# Autodesk Inventor assembly: Waffling60-MX
(part 2 of 2)
56. Open CASCADE STEP translator 7.5 468
57. Open CASCADE STEP translator 7.5 469
58. Open CASCADE STEP translator 7.5 470
59. Open CASCADE STEP translator 7.5 471
60. Open CASCADE STEP translator 7.5 472
61. Open CASCADE STEP translator 7.5 473
62. Open CASCADE STEP translator 7.5 474
63. Open CASCADE STEP translator 7.5 475
64. Open CASCADE STEP translator 7.5 476
65. Open CASCADE STEP translator 7.5 477
66. Open CASCADE STEP translator 7.5 478
67. Open CASCADE STEP translator 7.5 479
68. Open CASCADE STEP translator 7.5 480
69. Open CASCADE STEP translator 7.5 481
70. Open CASCADE STEP translator 7.5 482
71. Open CASCADE STEP translator 7.5 483
72. Open CASCADE STEP translator 7.5 484
73. Open CASCADE STEP translator 7.5 485
74. Open CASCADE STEP translator 7.5 486
75. Open CASCADE STEP translator 7.5 487
76. Open CASCADE STEP translator 7.5 488
77. Open CASCADE STEP translator 7.5 489
78. Open CASCADE STEP translator 7.5 490
79. Open CASCADE STEP translator 7.5 491
80. Open CASCADE STEP translator 7.5 492
81. Open CASCADE STEP translator 7.5 493
82. Open CASCADE STEP translator 7.5 494
83. Open CASCADE STEP translator 7.5 495
84. Open CASCADE STEP translator 7.5 496
85. Open CASCADE STEP translator 7.5 497
86. Open CASCADE STEP translator 7.5 498
87. Open CASCADE STEP translator 7.5 499
88. Open CASCADE STEP translator 7.5 500
89. Open CASCADE STEP translator 7.5 501
90. Open CASCADE STEP translator 7.5 502
91. Open CASCADE STEP translator 7.5 503
92. Open CASCADE STEP translator 7.5 504
93. Open CASCADE STEP translator 7.5 505
94. Open CASCADE STEP translator 7.5 506
95. Open CASCADE STEP translator 7.5 507
96. Open CASCADE STEP translator 7.5 508
97. Open CASCADE STEP translator 7.5 509
98. Open CASCADE STEP translator 7.5 510
99. Open CASCADE STEP translator 7.5 511
100. Open CASCADE STEP translator 7.5 512
101. Open CASCADE STEP translator 7.5 513
102. Open CASCADE STEP translator 7.5 514
103. Open CASCADE STEP translator 7.5 515
104. Open CASCADE STEP translator 7.5 516
105. Open CASCADE STEP translator 7.5 517
106. Open CASCADE STEP translator 7.5 518
107. Open CASCADE STEP translator 7.5 519
108. Open CASCADE STEP translator 7.5 520
109. Open CASCADE STEP translator 7.5 521
110. Open CASCADE STEP translator 7.5 522
111. Open CASCADE STEP translator 7.5 523
112. Open CASCADE STEP translator 7.5 524
113. Open CASCADE STEP translator 7.5 525
114. Open CASCADE STEP translator 7.5 526
115. Open CASCADE STEP translator 7.5 527
116. Open CASCADE STEP translator 7.5 528
117. Open CASCADE STEP translator 7.5 529
118. Open CASCADE STEP translator 7.5 530
119. Open CASCADE STEP translator 7.5 531
120. Open CASCADE STEP translator 7.5 532
121. Open CASCADE STEP translator 7.5 533
122. Open CASCADE STEP translator 7.5 534
123. Open CASCADE STEP translator 7.5 535
124. Open CASCADE STEP translator 7.5 536
125. Open CASCADE STEP translator 7.5 537
126. Open CASCADE STEP translator 7.5 538
127. Open CASCADE STEP translator 7.5 539
128. Open CASCADE STEP translator 7.5 540
129. Open CASCADE STEP translator 7.5 541
130. Open CASCADE STEP translator 7.5 542
131. Open CASCADE STEP translator 7.5 543
132. Open CASCADE STEP translator 7.5 544
133. Open CASCADE STEP translator 7.5 545
134. Open CASCADE STEP translator 7.5 546
135. Open CASCADE STEP translator 7.5 547
136. Open CASCADE STEP translator 7.5 548
137. Open CASCADE STEP translator 7.5 549
138. Open CASCADE STEP translator 7.5 550
139. Open CASCADE STEP translator 7.5 551
140. Open CASCADE STEP translator 7.5 552
141. Open CASCADE STEP translator 7.5 553
142. Open CASCADE STEP translator 7.5 554
143. Open CASCADE STEP translator 7.5 555
144. Open CASCADE STEP translator 7.5 556
145. Open CASCADE STEP translator 7.5 557
146. Open CASCADE STEP translator 7.5 558
147. Open CASCADE STEP translator 7.5 559
148. Open CASCADE STEP translator 7.5 560
149. Open CASCADE STEP translator 7.5 561
150. Open CASCADE STEP translator 7.5 562
151. Open CASCADE STEP translator 7.5 563
152. Open CASCADE STEP translator 7.5 564
153. Open CASCADE STEP translator 7.5 565
154. Open CASCADE STEP translator 7.5 566
155. Open CASCADE STEP translator 7.5 567
156. Open CASCADE STEP translator 7.5 568
157. Open CASCADE STEP translator 7.5 569
158. Open CASCADE STEP translator 7.5 570
159. Open CASCADE STEP translator 7.5 571
160. Open CASCADE STEP translator 7.5 572
161. Open CASCADE STEP translator 7.5 573
162. Open CASCADE STEP translator 7.5 574
163. Open CASCADE STEP translator 7.5 575
164. Open CASCADE STEP translator 7.5 576
165. Open CASCADE STEP translator 7.5 577
166. Open CASCADE STEP translator 7.5 578
167. Open CASCADE STEP translator 7.5 579
168. Open CASCADE STEP translator 7.5 580
169. Open CASCADE STEP translator 7.5 581
170. Open CASCADE STEP translator 7.5 582
171. Open CASCADE STEP translator 7.5 583
172. Open CASCADE STEP translator 7.5 584
173. Open CASCADE STEP translator 7.5 585
174. Open CASCADE STEP translator 7.5 586
175. Open CASCADE STEP translator 7.5 587
176. Open CASCADE STEP translator 7.5 588
177. Open CASCADE STEP translator 7.5 589
178. Open CASCADE STEP translator 7.5 590
179. Open CASCADE STEP translator 7.5 591
180. Open CASCADE STEP translator 7.5 592
181. Open CASCADE STEP translator 7.5 593
182. Open CASCADE STEP translator 7.5 594
183. Open CASCADE STEP translator 7.5 595
184. Open CASCADE STEP translator 7.5 596
185. Open CASCADE STEP translator 7.5 597
186. Open CASCADE STEP translator 7.5 598
187. Open CASCADE STEP translator 7.5 599
188. Open CASCADE STEP translator 7.5 600
189. Open CASCADE STEP translator 7.5 601
190. Open CASCADE STEP translator 7.5 602
191. Open CASCADE STEP translator 7.5 603
192. Open CASCADE STEP translator 7.5 604
193. Open CASCADE STEP translator 7.5 605
194. Open CASCADE STEP translator 7.5 606
195. Open CASCADE STEP translator 7.5 607
196. Open CASCADE STEP translator 7.5 608
197. Open CASCADE STEP translator 7.5 609
198. Open CASCADE STEP translator 7.5 610
199. Open CASCADE STEP translator 7.5 611
200. Open CASCADE STEP translator 7.5 612
201. Open CASCADE STEP translator 7.5 613
202. Open CASCADE STEP translator 7.5 614
203. Open CASCADE STEP translator 7.5 615
204. Open CASCADE STEP translator 7.5 616
205. Open CASCADE STEP translator 7.5 617
206. Open CASCADE STEP translator 7.5 618
207. Open CASCADE STEP translator 7.5 619
208. Open CASCADE STEP translator 7.5 620
209. Open CASCADE STEP translator 7.5 621
210. Open CASCADE STEP translator 7.5 622
211. Open CASCADE STEP translator 7.5 623
212. Open CASCADE STEP translator 7.5 624
213. Open CASCADE STEP translator 7.5 625
214. Open CASCADE STEP translator 7.5 626
215. Open CASCADE STEP translator 7.5 627
216. Open CASCADE STEP translator 7.5 628
217. Open CASCADE STEP translator 7.5 629
218. Open CASCADE STEP translator 7.5 630
219. Open CASCADE STEP translator 7.5 631
220. Open CASCADE STEP translator 7.5 632
221. Open CASCADE STEP translator 7.5 633
222. Open CASCADE STEP translator 7.5 634
223. Open CASCADE STEP translator 7.5 635
224. Open CASCADE STEP translator 7.5 636
225. Open CASCADE STEP translator 7.5 637
226. Open CASCADE STEP translator 7.5 638
227. Open CASCADE STEP translator 7.5 639
228. Open CASCADE STEP translator 7.5 640
229. Open CASCADE STEP translator 7.5 641
230. Open CASCADE STEP translator 7.5 642
231. Open CASCADE STEP translator 7.5 643
232. Open CASCADE STEP translator 7.5 644
233. Open CASCADE STEP translator 7.5 645
234. Open CASCADE STEP translator 7.5 646
235. Open CASCADE STEP translator 7.5 647
236. Open CASCADE STEP translator 7.5 648
237. Open CASCADE STEP translator 7.5 649
238. Open CASCADE STEP translator 7.5 650
239. Open CASCADE STEP translator 7.5 651
240. Open CASCADE STEP translator 7.5 652
241. Open CASCADE STEP translator 7.5 653
242. Open CASCADE STEP translator 7.5 654
243. Open CASCADE STEP translator 7.5 655
244. Open CASCADE STEP translator 7.5 656
245. Open CASCADE STEP translator 7.5 657
246. Open CASCADE STEP translator 7.5 658
247. Open CASCADE STEP translator 7.5 659
248. Open CASCADE STEP translator 7.5 660
249. Open CASCADE STEP translator 7.5 661
250. Open CASCADE STEP translator 7.5 662
251. Open CASCADE STEP translator 7.5 663
252. Open CASCADE STEP translator 7.5 664
253. Open CASCADE STEP translator 7.5 665
254. Open CASCADE STEP translator 7.5 666
255. Open CASCADE STEP translator 7.5 667
256. Open CASCADE STEP translator 7.5 668
257. Open CASCADE STEP translator 7.5 669
258. Open CASCADE STEP translator 7.5 670
259. Open CASCADE STEP translator 7.5 671
260. Open CASCADE STEP translator 7.5 672
261. Open CASCADE STEP translator 7.5 673
262. Open CASCADE STEP translator 7.5 674
263. Open CASCADE STEP translator 7.5 675
264. Open CASCADE STEP translator 7.5 676
265. Open CASCADE STEP translator 7.5 677
266. Open CASCADE STEP translator 7.5 678
267. Open CASCADE STEP translator 7.5 679
268. Open CASCADE STEP translator 7.5 680
269. Open CASCADE STEP translator 7.5 681
270. Open CASCADE STEP translator 7.5 682
271. Open CASCADE STEP translator 7.5 683
272. Open CASCADE STEP translator 7.5 684
273. Open CASCADE STEP translator 7.5 685
274. Open CASCADE STEP translator 7.5 686
275. Open CASCADE STEP translator 7.5 687
276. Open CASCADE STEP translator 7.5 688
277. Open CASCADE STEP translator 7.5 689
278. Open CASCADE STEP translator 7.5 690
279. Open CASCADE STEP translator 7.5 691
280. Open CASCADE STEP translator 7.5 692
281. Open CASCADE STEP translator 7.5 693
282. Open CASCADE STEP translator 7.5 694
283. Open CASCADE STEP translator 7.5 695
284. Open CASCADE STEP translator 7.5 696
285. Open CASCADE STEP translator 7.5 697
286. Open CASCADE STEP translator 7.5 698
287. Open CASCADE STEP translator 7.5 699
288. Open CASCADE STEP translator 7.5 700
289. Open CASCADE STEP translator 7.5 701
290. Open CASCADE STEP translator 7.5 702
291. Open CASCADE STEP translator 7.5 703
292. Open CASCADE STEP translator 7.5 704
293. Open CASCADE STEP translator 7.5 705
294. Open CASCADE STEP translator 7.5 706
295. Open CASCADE STEP translator 7.5 707
296. Open CASCADE STEP translator 7.5 708
297. Open CASCADE STEP translator 7.5 709
298. Open CASCADE STEP translator 7.5 710
299. Open CASCADE STEP translator 7.5 711
300. Open CASCADE STEP translator 7.5 712
301. Open CASCADE STEP translator 7.5 713
302. Open CASCADE STEP translator 7.5 714
303. Open CASCADE STEP translator 7.5 715
304. Open CASCADE STEP translator 7.5 716
305. Open CASCADE STEP translator 7.5 717
306. Open CASCADE STEP translator 7.5 718
307. Open CASCADE STEP translator 7.5 719
308. Open CASCADE STEP translator 7.5 720
309. Open CASCADE STEP translator 7.5 721
310. Open CASCADE STEP translator 7.5 722
311. Open CASCADE STEP translator 7.5 723
312. Open CASCADE STEP translator 7.5 724
313. Open CASCADE STEP translator 7.5 725
314. Open CASCADE STEP translator 7.5 726
315. Open CASCADE STEP translator 7.5 727
316. Open CASCADE STEP translator 7.5 728
317. Open CASCADE STEP translator 7.5 729
318. Open CASCADE STEP translator 7.5 730
319. Open CASCADE STEP translator 7.5 731
320. Open CASCADE STEP translator 7.5 732
321. Open CASCADE STEP translator 7.5 733
322. Open CASCADE STEP translator 7.5 734
323. Open CASCADE STEP translator 7.5 735
324. Open CASCADE STEP translator 7.5 736
325. Open CASCADE STEP translator 7.5 737
326. Open CASCADE STEP translator 7.5 738
327. Open CASCADE STEP translator 7.5 739
328. Open CASCADE STEP translator 7.5 740
329. Open CASCADE STEP translator 7.5 741
330. Open CASCADE STEP translator 7.5 742
331. Open CASCADE STEP translator 7.5 743
332. Open CASCADE STEP translator 7.5 744
333. Open CASCADE STEP translator 7.5 745
334. Open CASCADE STEP translator 7.5 746
335. Open CASCADE STEP translator 7.5 747
336. Open CASCADE STEP translator 7.5 748
337. Open CASCADE STEP translator 7.5 749
338. Open CASCADE STEP translator 7.5 750
339. Open CASCADE STEP translator 7.5 751
340. Open CASCADE STEP translator 7.5 752
341. Open CASCADE STEP translator 7.5 753
342. Open CASCADE STEP translator 7.5 754
343. Open CASCADE STEP translator 7.5 755
344. Open CASCADE STEP translator 7.5 756
345. Open CASCADE STEP translator 7.5 757
346. Open CASCADE STEP translator 7.5 758
347. Open CASCADE STEP translator 7.5 759
348. Open CASCADE STEP translator 7.5 760
349. Open CASCADE STEP translator 7.5 761
350. Open CASCADE STEP translator 7.5 762
351. Open CASCADE STEP translator 7.5 763
352. Open CASCADE STEP translator 7.5 764
353. Open CASCADE STEP translator 7.5 765
354. Open CASCADE STEP translator 7.5 766
355. Open CASCADE STEP translator 7.5 767
356. Open CASCADE STEP translator 7.5 768
357. Open CASCADE STEP translator 7.5 769
358. Open CASCADE STEP translator 7.5 770
359. Open CASCADE STEP translator 7.5 771
360. Open CASCADE STEP translator 7.5 772
361. Open CASCADE STEP translator 7.5 773
362. Open CASCADE STEP translator 7.5 774
363. Open CASCADE STEP translator 7.5 775
364. Open CASCADE STEP translator 7.5 776
365. Open CASCADE STEP translator 7.5 777
366. Open CASCADE STEP translator 7.5 778
367. Open CASCADE STEP translator 7.5 779
368. Open CASCADE STEP translator 7.5 780
369. Open CASCADE STEP translator 7.5 781
370. Open CASCADE STEP translator 7.5 782
371. Open CASCADE STEP translator 7.5 783
372. Open CASCADE STEP translator 7.5 784
373. Open CASCADE STEP translator 7.5 785
374. Open CASCADE STEP translator 7.5 786
375. Open CASCADE STEP translator 7.5 787
376. Open CASCADE STEP translator 7.5 788
377. Open CASCADE STEP translator 7.5 789
378. Open CASCADE STEP translator 7.5 790
379. Open CASCADE STEP translator 7.5 791
380. Open CASCADE STEP translator 7.5 792
381. Open CASCADE STEP translator 7.5 793
382. Open CASCADE STEP translator 7.5 794
383. Open CASCADE STEP translator 7.5 795
384. Open CASCADE STEP translator 7.5 796
385. Open CASCADE STEP translator 7.5 797
386. Open CASCADE STEP translator 7.5 798
387. Open CASCADE STEP translator 7.5 799
388. Open CASCADE STEP translator 7.5 800
389. Open CASCADE STEP translator 7.5 801
390. Open CASCADE STEP translator 7.5 802
391. Open CASCADE STEP translator 7.5 803
392. Open CASCADE STEP translator 7.5 804
393. Open CASCADE STEP translator 7.5 805
394. Open CASCADE STEP translator 7.5 806
395. Open CASCADE STEP translator 7.5 807
396. Open CASCADE STEP translator 7.5 808
397. Open CASCADE STEP translator 7.5 809
398. Open CASCADE STEP translator 7.5 810
399. Open CASCADE STEP translator 7.5 811
400. Open CASCADE STEP translator 7.5 812
401. Open CASCADE STEP translator 7.5 813
402. Open CASCADE STEP translator 7.5 814
403. Open CASCADE STEP translator 7.5 815
404. Open CASCADE STEP translator 7.5 816
405. Open CASCADE STEP translator 7.5 817
406. Open CASCADE STEP translator 7.5 818
407. Open CASCADE STEP translator 7.5 819
408. Open CASCADE STEP translator 7.5 820
409. Open CASCADE STEP translator 7.5 821
410. Open CASCADE STEP translator 7.5 822
411. Open CASCADE STEP translator 7.5 823
412. Open CASCADE STEP translator 7.5 824
## Named parameters: Finish1_Area = 278.887, Finish2_Area = 630.792
note: some values were not read from the file. Shown as the stored number, unit unknown: "Finish1_Area", "Finish2_Area".
